# Autodesk Inventor assembly: s-assy-shooter_frame
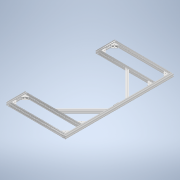
[picture p0: Inventor's stored thumbnail of the model, 180x180]
Saved by Autodesk Inventor 2022 (Build 260153000, 153)
## iProperties
Created: 2021-09-11
Part Number: s-assy-shooter_frame
Document SubType Name: Assembly
Designer: yuto6
Author: yuto6
## Documents named in this file (10)
- C:\Users\yuto6\Box\Public_Share\キャチロボバトルコンテスト2021\CAD\catchrobo_hardware\assy-shooter\s-assy-shooter_frame.iam
- C:\Users\yuto6\Box\Public_Share\キャチロボバトルコンテスト2021\CAD\catchrobo_hardware\assy-shooter\HFS5-2020-402_5.ipt
- C:\Users\yuto6\Box\Public_Share\キャチロボバトルコンテスト2021\CAD\catchrobo_hardware\assy-shooter\HPTBD5-SEP_b_.ipt
- C:\Users\yuto6\Box\Public_Share\キャチロボバトルコンテスト2021\CAD\catchrobo_hardware\assy-shooter\AIS2020_D\HNTP5-5.ipt
- C:\Users\yuto6\Box\Public_Share\キャチロボバトルコンテスト2021\CAD\catchrobo_hardware\assy-shooter\AIS2020_D\CBM5-8.ipt
- C:\Users\yuto6\Box\Public_Share\キャチロボバトルコンテスト2021\CAD\catchrobo_hardware\assy-robot\KNFS5-2020-2.ipt
- C:\Users\yuto6\Box\Public_Share\キャチロボバトルコンテスト2021\CAD\catchrobo_hardware\assy-robot\KNFS5-2020-3.ipt
- C:\Users\yuto6\Box\Public_Share\キャチロボバトルコンテスト2021\CAD\catchrobo_hardware\assy-shooter\HFBL5-2020-200.iam
- C:\Users\yuto6\Box\Public_Share\キャチロボバトルコンテスト2021\CAD\catchrobo_hardware\assy-shooter\HBLFSNK5-C-SEP.iam
- C:\Users\yuto6\Box\Public_Share\キャチロボバトルコンテスト2021\CAD\catchrobo_hardware\assy-shooter\s-assy-frame_bolt.iam
## Components (31 placed, 9 different names)
1. HFS5-2020-402_5:1 — メイト:1, メイト:2, フラッシュ:1, フラッシュ:2, メイト:6, メイト:8, メイト:13, メイト:14, フラッシュ:3, フラッシュ:4, メイト:21, フラッシュ:8, メイト:24, メイト:30, フラッシュ:16, メイト:37, メイト:40
2. HFS5-2020-402_5:2 — メイト:4, メイト:5, フラッシュ:1, フラッシュ:2, メイト:6, メイト:15, メイト:16, フラッシュ:5, フラッシュ:6, メイト:22, フラッシュ:7, メイト:23, メイト:28, メイト:34, フラッシュ:19, メイト:36, 角度:1, メイト:49, 角度:2, メイト:51
3. HPTBD5-SEP_b_:1 — メイト:3, メイト:7, メイト:8, メイト:9, メイト:10, メイト:11, メイト:12, メイト:19, メイト:20
4. HNTP5-5:2 — メイト:1, メイト:2, メイト:3
5. HNTP5-5:3 — メイト:4, メイト:5, メイト:7
6. CBM5-8:1 — メイト:9, メイト:11
7. CBM5-8:2 — メイト:10, メイト:12
8. HNTP5-5:4 — メイト:13, メイト:14, メイト:17
9. HNTP5-5:5 — メイト:15, メイト:16, メイト:18
10. CBM5-8:3 — メイト:17, メイト:20
11. CBM5-8:4 — メイト:18, メイト:19
12. KNFS5-2020-2:1 — フラッシュ:5, フラッシュ:6, メイト:22, フラッシュ:9, フラッシュ:10, メイト:25, メイト:33, フラッシュ:18, メイト:47
13. KNFS5-2020-2:2 — フラッシュ:3, フラッシュ:4, メイト:21, フラッシュ:12, フラッシュ:13, メイト:26, フラッシュ:21, メイト:39, メイト:42
14. KNFS5-2020-2:3 — フラッシュ:7, メイト:23, フラッシュ:11, フラッシュ:15, メイト:27, メイト:35, フラッシュ:24, メイト:45, 角度:3
15. KNFS5-2020-2:4 — フラッシュ:8, メイト:24, フラッシュ:14, メイト:29, フラッシュ:20, メイト:38, メイト:43, 角度:4
16. KNFS5-2020-3:1 — フラッシュ:9, フラッシュ:10, メイト:25, フラッシュ:11, メイト:46, フラッシュ:25, メイト:48
17. KNFS5-2020-3:2 — フラッシュ:12, フラッシュ:13, メイト:26, フラッシュ:14, フラッシュ:22, メイト:41, フラッシュ:23, メイト:44
18. HFBL5-2020-200:1 [sub-assembly] — フラッシュ:15, メイト:27, メイト:28, メイト:52, メイト:53
19. HFBL5-2020-200:2 [sub-assembly] — メイト:29, メイト:30, フラッシュ:16, メイト:50, メイト:54
20. HBLFSNK5-C-SEP:2 [sub-assembly] — メイト:33, フラッシュ:18, メイト:34
21. HBLFSNK5-C-SEP:3 [sub-assembly] — フラッシュ:19, メイト:35, メイト:36, フラッシュ:26
22. HBLFSNK5-C-SEP:4 [sub-assembly] — フラッシュ:20, メイト:37, メイト:38, フラッシュ:27
23. HBLFSNK5-C-SEP:5 [sub-assembly] — フラッシュ:21, メイト:39, メイト:40
24. HBLFSNK5-C-SEP:6 [sub-assembly] — フラッシュ:25, メイト:47, メイト:48
25. HBLFSNK5-C-SEP:7 [sub-assembly] — フラッシュ:24, メイト:45, メイト:46
26. HBLFSNK5-C-SEP:8 [sub-assembly] — フラッシュ:22, メイト:41, メイト:42
27. HBLFSNK5-C-SEP:9 [sub-assembly] — フラッシュ:23, メイト:43, メイト:44
28. s-assy-frame_bolt:1 [sub-assembly] — 角度:1, メイト:49, メイト:50
29. s-assy-frame_bolt:2 [sub-assembly] — 角度:2, メイト:51, メイト:52
30. s-assy-frame_bolt:3 [sub-assembly] — フラッシュ:26, 角度:3, メイト:53
31. s-assy-frame_bolt:4 [sub-assembly] — 角度:4, フラッシュ:27, メイト:54
## Relationships (82: Mate 52, Flush 26, Angle 4)
- メイト:1 [Mate]: HFS5-2020-402_5:1 ↔ HNTP5-5:2
- メイト:2 [Mate]: HFS5-2020-402_5:1 ↔ HNTP5-5:2
- メイト:3 [Mate]: HPTBD5-SEP_b_:1 ↔ HNTP5-5:2
- メイト:4 [Mate]: HFS5-2020-402_5:2 ↔ HNTP5-5:3
- メイト:5 [Mate]: HFS5-2020-402_5:2 ↔ HNTP5-5:3
- フラッシュ:1 [Flush]: HFS5-2020-402_5:1 ↔ HFS5-2020-402_5:2
- フラッシュ:2 [Flush]: HFS5-2020-402_5:1 ↔ HFS5-2020-402_5:2
- メイト:6 [Mate]: HFS5-2020-402_5:1 ↔ HFS5-2020-402_5:2
- メイト:7 [Mate]: HPTBD5-SEP_b_:1 ↔ HNTP5-5:3
- メイト:8 [Mate]: HFS5-2020-402_5:1 ↔ HPTBD5-SEP_b_:1
- メイト:9 [Mate]: HPTBD5-SEP_b_:1 ↔ CBM5-8:1
- メイト:10 [Mate]: HPTBD5-SEP_b_:1 ↔ CBM5-8:2
- メイト:11 [Mate]: HPTBD5-SEP_b_:1 ↔ CBM5-8:1
- メイト:12 [Mate]: HPTBD5-SEP_b_:1 ↔ CBM5-8:2
- メイト:13 [Mate]: HFS5-2020-402_5:1 ↔ HNTP5-5:4
- メイト:14 [Mate]: HFS5-2020-402_5:1 ↔ HNTP5-5:4
- メイト:15 [Mate]: HFS5-2020-402_5:2 ↔ HNTP5-5:5
- メイト:16 [Mate]: HFS5-2020-402_5:2 ↔ HNTP5-5:5
- メイト:17 [Mate]: HNTP5-5:4 ↔ CBM5-8:3
- メイト:18 [Mate]: HNTP5-5:5 ↔ CBM5-8:4
- メイト:19 [Mate]: HPTBD5-SEP_b_:1 ↔ CBM5-8:4
- メイト:20 [Mate]: HPTBD5-SEP_b_:1 ↔ CBM5-8:3
- フラッシュ:3 [Flush]: HFS5-2020-402_5:1 ↔ KNFS5-2020-2:2
- フラッシュ:4 [Flush]: HFS5-2020-402_5:1 ↔ KNFS5-2020-2:2
- メイト:21 [Mate]: HFS5-2020-402_5:1 ↔ KNFS5-2020-2:2
- フラッシュ:5 [Flush]: HFS5-2020-402_5:2 ↔ KNFS5-2020-2:1
- フラッシュ:6 [Flush]: HFS5-2020-402_5:2 ↔ KNFS5-2020-2:1
- メイト:22 [Mate]: HFS5-2020-402_5:2 ↔ KNFS5-2020-2:1
- フラッシュ:7 [Flush]: HFS5-2020-402_5:2 ↔ KNFS5-2020-2:3
- メイト:23 [Mate]: HFS5-2020-402_5:2 ↔ KNFS5-2020-2:3
- フラッシュ:8 [Flush]: HFS5-2020-402_5:1 ↔ KNFS5-2020-2:4
- メイト:24 [Mate]: HFS5-2020-402_5:1 ↔ KNFS5-2020-2:4
- フラッシュ:9 [Flush]: KNFS5-2020-2:1 ↔ KNFS5-2020-3:1
- フラッシュ:10 [Flush]: KNFS5-2020-2:1 ↔ KNFS5-2020-3:1
- メイト:25 [Mate]: KNFS5-2020-2:1 ↔ KNFS5-2020-3:1
- フラッシュ:11 [Flush]: KNFS5-2020-2:3 ↔ KNFS5-2020-3:1
- フラッシュ:12 [Flush]: KNFS5-2020-2:2 ↔ KNFS5-2020-3:2
- フラッシュ:13 [Flush]: KNFS5-2020-2:2 ↔ KNFS5-2020-3:2
- メイト:26 [Mate]: KNFS5-2020-2:2 ↔ KNFS5-2020-3:2
- フラッシュ:14 [Flush]: KNFS5-2020-2:4 ↔ KNFS5-2020-3:2
- フラッシュ:15 [Flush]: KNFS5-2020-2:3 ↔ HFBL5-2020-200:1
- メイト:27 [Mate]: KNFS5-2020-2:3 ↔ HFBL5-2020-200:1
- メイト:28 [Mate]: HFS5-2020-402_5:2 ↔ HFBL5-2020-200:1
- メイト:29 [Mate]: KNFS5-2020-2:4 ↔ HFBL5-2020-200:2
- メイト:30 [Mate]: HFS5-2020-402_5:1 ↔ HFBL5-2020-200:2
- フラッシュ:16 [Flush]: HFS5-2020-402_5:1 ↔ HFBL5-2020-200:2
- メイト:33 [Mate]: KNFS5-2020-2:1 ↔ HBLFSNK5-C-SEP:2
- フラッシュ:18 [Flush]: KNFS5-2020-2:1 ↔ HBLFSNK5-C-SEP:2
- メイト:34 [Mate]: HFS5-2020-402_5:2 ↔ HBLFSNK5-C-SEP:2
- フラッシュ:19 [Flush]: HFS5-2020-402_5:2 ↔ HBLFSNK5-C-SEP:3
- メイト:35 [Mate]: KNFS5-2020-2:3 ↔ HBLFSNK5-C-SEP:3
- メイト:36 [Mate]: HFS5-2020-402_5:2 ↔ HBLFSNK5-C-SEP:3
- フラッシュ:20 [Flush]: KNFS5-2020-2:4 ↔ HBLFSNK5-C-SEP:4
- メイト:37 [Mate]: HFS5-2020-402_5:1 ↔ HBLFSNK5-C-SEP:4
- メイト:38 [Mate]: KNFS5-2020-2:4 ↔ HBLFSNK5-C-SEP:4
- フラッシュ:21 [Flush]: KNFS5-2020-2:2 ↔ HBLFSNK5-C-SEP:5
- メイト:39 [Mate]: KNFS5-2020-2:2 ↔ HBLFSNK5-C-SEP:5
- メイト:40 [Mate]: HFS5-2020-402_5:1 ↔ HBLFSNK5-C-SEP:5
- フラッシュ:22 [Flush]: KNFS5-2020-3:2 ↔ HBLFSNK5-C-SEP:8
- メイト:41 [Mate]: KNFS5-2020-3:2 ↔ HBLFSNK5-C-SEP:8
- メイト:42 [Mate]: KNFS5-2020-2:2 ↔ HBLFSNK5-C-SEP:8
- フラッシュ:23 [Flush]: KNFS5-2020-3:2 ↔ HBLFSNK5-C-SEP:9
- メイト:43 [Mate]: KNFS5-2020-2:4 ↔ HBLFSNK5-C-SEP:9
- メイト:44 [Mate]: KNFS5-2020-3:2 ↔ HBLFSNK5-C-SEP:9
- フラッシュ:24 [Flush]: KNFS5-2020-2:3 ↔ HBLFSNK5-C-SEP:7
- メイト:45 [Mate]: KNFS5-2020-2:3 ↔ HBLFSNK5-C-SEP:7
- メイト:46 [Mate]: KNFS5-2020-3:1 ↔ HBLFSNK5-C-SEP:7
- フラッシュ:25 [Flush]: KNFS5-2020-3:1 ↔ HBLFSNK5-C-SEP:6
- メイト:47 [Mate]: KNFS5-2020-2:1 ↔ HBLFSNK5-C-SEP:6
- メイト:48 [Mate]: KNFS5-2020-3:1 ↔ HBLFSNK5-C-SEP:6
- 角度:1 [Angle] (0 deg): HFS5-2020-402_5:2 ↔ s-assy-frame_bolt:1
- メイト:49 [Mate]: HFS5-2020-402_5:2 ↔ s-assy-frame_bolt:1
- メイト:50 [Mate]: HFBL5-2020-200:2 ↔ s-assy-frame_bolt:1
- 角度:2 [Angle] (0 deg): HFS5-2020-402_5:2 ↔ s-assy-frame_bolt:2
- メイト:51 [Mate]: HFS5-2020-402_5:2 ↔ s-assy-frame_bolt:2
- メイト:52 [Mate]: HFBL5-2020-200:1 ↔ s-assy-frame_bolt:2
- フラッシュ:26 [Flush]: HBLFSNK5-C-SEP:3 ↔ s-assy-frame_bolt:3
- 角度:3 [Angle] (0 deg): KNFS5-2020-2:3 ↔ s-assy-frame_bolt:3
- メイト:53 [Mate]: HFBL5-2020-200:1 ↔ s-assy-frame_bolt:3
- 角度:4 [Angle] (0 deg): KNFS5-2020-2:4 ↔ s-assy-frame_bolt:4
- フラッシュ:27 [Flush]: HBLFSNK5-C-SEP:4 ↔ s-assy-frame_bolt:4
- メイト:54 [Mate]: HFBL5-2020-200:2 ↔ s-assy-frame_bolt:4
